# Autodesk Inventor assembly: MR106ZZ1
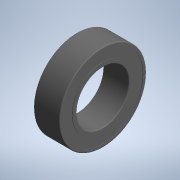
[picture p0: Inventor's stored thumbnail of the model, 180x180]
Saved by Autodesk Inventor 2022 (Build 260153000, 153)
## iProperties
Category: PARTsolutions
Company: NSK_RB
Part Number: MR106ZZ1
Catalog Web Link: www.cadenas.de
Description: Shielded Type ZZ-ZZS-
Vendor: NSK_RB
Document SubType Name: Assembly
Designer: partserver
Manufacturer: NSK_RB
Mass: 0.68 g
Surface Area: 5.5525 cm^2
Volume: 0.0980642 cm^3
Density: 6.93423 g/cm^3
PSOL_IDENT_0: {$CADENAS_DATA\23d-libs\nsk_rb\roller_bearings\deep_groove_bb\exstra_small_miniatur_bb\metric_design
PSOL_IDENT_1: \shielded_type_zz_zzs_asmtab.prj},176 {VTYP=3D},{STYP=ASSTAB},{NB=MR106ZZ1},{LINA=MR106ZZ1},{NN=Shie
PSOL_IDENT_2: lded Type ZZ-ZZS},{DATE=25.05.2021 06:41:25},{GEOMDATE=14.01.2008},{VERSION=},{LINEID=600},{WBVAR=},
PSOL_IDENT_3: {WBNUMERIC=}  {NB=MR106ZZ1},{LINA=MR106ZZ1},{KT=DUMMY},{IDNR=},{STAN=Standard},{ORDER=MR106ZZ1},{SD=
PSOL_IDENT_4: 6.0},{X=6.0},{DI1=7.04},{DI2=7.04},{SDE1=8.90},{SDE2=9.25},{D=10},{DD=10},{B=0.0},{B1=3.0},{R=0.00},
PSOL_IDENT_5: {R1=0.10},{CR1=495},{COR1=218},{CR2=51},{COR2=22.0},{LG=45000},{LO=53000},{DA=0.0},{DB=7.0},{DA1=0.0
PSOL_IDENT_6: },{DB1=9.3},{RA=0.00},{RB=0.10},{MASS=0.68},{SC=1},{PPATH=shielded_type_zz_zzs_asmtpl.prj}
NB: MR106ZZ1
NN: Shielded Type ZZ-ZZS
NBSYN: $ORDER.
LINA: MR106ZZ1
CATALOG: NSK Rolling Bearing
STAN: Standard
ORDER: MR106ZZ1
SD: 6
D: 10
B1: 3
R1: 0.1
CR1: 495
COR1: 218
CR2: 51
COR2: 22
LG: 45000
DB: 7
DB1: 9.3
RB: 0.1
MASS: 0.68
SUPPLIER: NSK_RB
ARTICLENO: MR106ZZ1
BOMINFO: MR106ZZ1
CREATOR: CADENAS GmbH
Title: MR106ZZ1
Author: Cadenas PARTsolutions
## Documents named in this file (6)
- C:\Users\rkawaba1\Documents\GrabCAD\NHK2022\BasicParts\Bearing\MR106ZZ1\MR106ZZ1.iam
- C:\Users\rkawaba1\Documents\GrabCAD\NHK2022\BasicParts\Bearing\MR106ZZ1\MR106ZZ1 Outer Ring.ipt
- C:\Users\rkawaba1\Documents\GrabCAD\NHK2022\BasicParts\Bearing\MR106ZZ1\MR106ZZ1 Inner Ring.ipt
- C:\Users\rkawaba1\Documents\GrabCAD\NHK2022\BasicParts\Bearing\MR106ZZ1\MR106ZZ1 Shield1.ipt
- C:\Users\rkawaba1\Documents\GrabCAD\NHK2022\BasicParts\Bearing\MR106ZZ1\MR106ZZ1 Ball.ipt
- C:\Users\rkawaba1\Documents\GrabCAD\NHK2022\BasicParts\Bearing\MR106ZZ1\MR106ZZ1 Shield2.ipt
## Components (20 placed, 5 different names)
1. MR106ZZ1 Outer Ring:1 — ip_st_or_1_XY@1 <-> ip_st_ir_1a_XY@2, ip_st_or_1_Z@1 <-> ip_st_ir_1a_Z@2, ip_st_or_1_YZ@1 <-> ip_st_ir_1a_YZ@2, ip_st_or_2_XY@1 <-> ip_st_s2_XY@20, ip_st_or_2_Z@1 <-> ip_st_s2_Z@20, ip_st_or_2_YZ@1 <-> ip_st_s2_YZ@20
2. MR106ZZ1 Inner Ring:1 — ip_st_or_1_XY@1 <-> ip_st_ir_1a_XY@2, ip_st_or_1_Z@1 <-> ip_st_ir_1a_Z@2, ip_st_or_1_YZ@1 <-> ip_st_ir_1a_YZ@2, ip_st_ir_2a_XY@2 <-> ip_st_s1_XY@3, ip_st_ir_2a_Z@2 <-> ip_st_s1_Z@3, ip_st_ir_2a_YZ@2 <-> ip_st_s1_YZ@3, ip_st_ir_1_1_XY@2 <-> ip_st_b_XY@4, ip_st_ir_1_1_Z@2 <-> ip_st_b_Z@4, ip_st_ir_1_1_YZ@2 <-> ip_st_b_YZ@4, ip_st_ir_1_2_XY@2 <-> ip_st_b_XY@5, ip_st_ir_1_2_Z@2 <-> ip_st_b_Z@5, ip_st_ir_1_2_YZ@2 <-> ip_st_b_YZ@5, ip_st_ir_1_3_XY@2 <-> ip_st_b_XY@6, ip_st_ir_1_3_Z@2 <-> ip_st_b_Z@6, ip_st_ir_1_3_YZ@2 <-> ip_st_b_YZ@6, ip_st_ir_1_4_XY@2 <-> ip_st_b_XY@7, ip_st_ir_1_4_Z@2 <-> ip_st_b_Z@7, ip_st_ir_1_4_YZ@2 <-> ip_st_b_YZ@7, ip_st_ir_1_5_XY@2 <-> ip_st_b_XY@8, ip_st_ir_1_5_Z@2 <-> ip_st_b_Z@8, ip_st_ir_1_5_YZ@2 <-> ip_st_b_YZ@8, ip_st_ir_1_6_XY@2 <-> ip_st_b_XY@9, ip_st_ir_1_6_Z@2 <-> ip_st_b_Z@9, ip_st_ir_1_6_YZ@2 <-> ip_st_b_YZ@9, ip_st_ir_1_7_XY@2 <-> ip_st_b_XY@10, ip_st_ir_1_7_Z@2 <-> ip_st_b_Z@10, ip_st_ir_1_7_YZ@2 <-> ip_st_b_YZ@10, ip_st_ir_1_8_XY@2 <-> ip_st_b_XY@11, ip_st_ir_1_8_Z@2 <-> ip_st_b_Z@11, ip_st_ir_1_8_YZ@2 <-> ip_st_b_YZ@11, ip_st_ir_1_9_XY@2 <-> ip_st_b_XY@12, ip_st_ir_1_9_Z@2 <-> ip_st_b_Z@12, ip_st_ir_1_9_YZ@2 <-> ip_st_b_YZ@12, ip_st_ir_1_10_XY@2 <-> ip_st_b_XY@13, ip_st_ir_1_10_Z@2 <-> ip_st_b_Z@13, ip_st_ir_1_10_YZ@2 <-> ip_st_b_YZ@13, ip_st_ir_1_11_XY@2 <-> ip_st_b_XY@14, ip_st_ir_1_11_Z@2 <-> ip_st_b_Z@14, ip_st_ir_1_11_YZ@2 <-> ip_st_b_YZ@14, ip_st_ir_1_12_XY@2 <-> ip_st_b_XY@15, ip_st_ir_1_12_Z@2 <-> ip_st_b_Z@15, ip_st_ir_1_12_YZ@2 <-> ip_st_b_YZ@15, ip_st_ir_1_13_XY@2 <-> ip_st_b_XY@16, ip_st_ir_1_13_Z@2 <-> ip_st_b_Z@16, ip_st_ir_1_13_YZ@2 <-> ip_st_b_YZ@16, ip_st_ir_1_14_XY@2 <-> ip_st_b_XY@17, ip_st_ir_1_14_Z@2 <-> ip_st_b_Z@17, ip_st_ir_1_14_YZ@2 <-> ip_st_b_YZ@17, ip_st_ir_1_15_XY@2 <-> ip_st_b_XY@18, ip_st_ir_1_15_Z@2 <-> ip_st_b_Z@18, ip_st_ir_1_15_YZ@2 <-> ip_st_b_YZ@18, ip_st_ir_1_16_XY@2 <-> ip_st_b_XY@19, ip_st_ir_1_16_Z@2 <-> ip_st_b_Z@19, ip_st_ir_1_16_YZ@2 <-> ip_st_b_YZ@19
3. MR106ZZ1 Shield1:1 — ip_st_ir_2a_XY@2 <-> ip_st_s1_XY@3, ip_st_ir_2a_Z@2 <-> ip_st_s1_Z@3, ip_st_ir_2a_YZ@2 <-> ip_st_s1_YZ@3
4. MR106ZZ1 Ball:1 — ip_st_ir_1_1_XY@2 <-> ip_st_b_XY@4, ip_st_ir_1_1_Z@2 <-> ip_st_b_Z@4, ip_st_ir_1_1_YZ@2 <-> ip_st_b_YZ@4
5. MR106ZZ1 Ball:2 — ip_st_ir_1_2_XY@2 <-> ip_st_b_XY@5, ip_st_ir_1_2_Z@2 <-> ip_st_b_Z@5, ip_st_ir_1_2_YZ@2 <-> ip_st_b_YZ@5
6. MR106ZZ1 Ball:3 — ip_st_ir_1_3_XY@2 <-> ip_st_b_XY@6, ip_st_ir_1_3_Z@2 <-> ip_st_b_Z@6, ip_st_ir_1_3_YZ@2 <-> ip_st_b_YZ@6
7. MR106ZZ1 Ball:4 — ip_st_ir_1_4_XY@2 <-> ip_st_b_XY@7, ip_st_ir_1_4_Z@2 <-> ip_st_b_Z@7, ip_st_ir_1_4_YZ@2 <-> ip_st_b_YZ@7
8. MR106ZZ1 Ball:5 — ip_st_ir_1_5_XY@2 <-> ip_st_b_XY@8, ip_st_ir_1_5_Z@2 <-> ip_st_b_Z@8, ip_st_ir_1_5_YZ@2 <-> ip_st_b_YZ@8
9. MR106ZZ1 Ball:6 — ip_st_ir_1_6_XY@2 <-> ip_st_b_XY@9, ip_st_ir_1_6_Z@2 <-> ip_st_b_Z@9, ip_st_ir_1_6_YZ@2 <-> ip_st_b_YZ@9
10. MR106ZZ1 Ball:7 — ip_st_ir_1_7_XY@2 <-> ip_st_b_XY@10, ip_st_ir_1_7_Z@2 <-> ip_st_b_Z@10, ip_st_ir_1_7_YZ@2 <-> ip_st_b_YZ@10
11. MR106ZZ1 Ball:8 — ip_st_ir_1_8_XY@2 <-> ip_st_b_XY@11, ip_st_ir_1_8_Z@2 <-> ip_st_b_Z@11, ip_st_ir_1_8_YZ@2 <-> ip_st_b_YZ@11
12. MR106ZZ1 Ball:9 — ip_st_ir_1_9_XY@2 <-> ip_st_b_XY@12, ip_st_ir_1_9_Z@2 <-> ip_st_b_Z@12, ip_st_ir_1_9_YZ@2 <-> ip_st_b_YZ@12
13. MR106ZZ1 Ball:10 — ip_st_ir_1_10_XY@2 <-> ip_st_b_XY@13, ip_st_ir_1_10_Z@2 <-> ip_st_b_Z@13, ip_st_ir_1_10_YZ@2 <-> ip_st_b_YZ@13
14. MR106ZZ1 Ball:11 — ip_st_ir_1_11_XY@2 <-> ip_st_b_XY@14, ip_st_ir_1_11_Z@2 <-> ip_st_b_Z@14, ip_st_ir_1_11_YZ@2 <-> ip_st_b_YZ@14
15. MR106ZZ1 Ball:12 — ip_st_ir_1_12_XY@2 <-> ip_st_b_XY@15, ip_st_ir_1_12_Z@2 <-> ip_st_b_Z@15, ip_st_ir_1_12_YZ@2 <-> ip_st_b_YZ@15
16. MR106ZZ1 Ball:13 — ip_st_ir_1_13_XY@2 <-> ip_st_b_XY@16, ip_st_ir_1_13_Z@2 <-> ip_st_b_Z@16, ip_st_ir_1_13_YZ@2 <-> ip_st_b_YZ@16
17. MR106ZZ1 Ball:14 — ip_st_ir_1_14_XY@2 <-> ip_st_b_XY@17, ip_st_ir_1_14_Z@2 <-> ip_st_b_Z@17, ip_st_ir_1_14_YZ@2 <-> ip_st_b_YZ@17
18. MR106ZZ1 Ball:15 — ip_st_ir_1_15_XY@2 <-> ip_st_b_XY@18, ip_st_ir_1_15_Z@2 <-> ip_st_b_Z@18, ip_st_ir_1_15_YZ@2 <-> ip_st_b_YZ@18
19. MR106ZZ1 Ball:16 — ip_st_ir_1_16_XY@2 <-> ip_st_b_XY@19, ip_st_ir_1_16_Z@2 <-> ip_st_b_Z@19, ip_st_ir_1_16_YZ@2 <-> ip_st_b_YZ@19
20. MR106ZZ1 Shield2:1 — ip_st_or_2_XY@1 <-> ip_st_s2_XY@20, ip_st_or_2_Z@1 <-> ip_st_s2_Z@20, ip_st_or_2_YZ@1 <-> ip_st_s2_YZ@20
## Relationships (57: Mate 37, Angle 19, Flush 1)
- ip_st_or_1_XY@1 <-> ip_st_ir_1a_XY@2 [Flush]: MR106ZZ1 Outer Ring:1 ↔ MR106ZZ1 Inner Ring:1
- ip_st_or_1_Z@1 <-> ip_st_ir_1a_Z@2 [Mate]: MR106ZZ1 Outer Ring:1 ↔ MR106ZZ1 Inner Ring:1
- ip_st_or_1_YZ@1 <-> ip_st_ir_1a_YZ@2 [Angle] (90 deg): MR106ZZ1 Outer Ring:1 ↔ MR106ZZ1 Inner Ring:1
- ip_st_ir_2a_XY@2 <-> ip_st_s1_XY@3 [Mate]: MR106ZZ1 Inner Ring:1 ↔ MR106ZZ1 Shield1:1
- ip_st_ir_2a_Z@2 <-> ip_st_s1_Z@3 [Mate]: MR106ZZ1 Inner Ring:1 ↔ MR106ZZ1 Shield1:1
- ip_st_ir_2a_YZ@2 <-> ip_st_s1_YZ@3 [Angle] (0 deg): MR106ZZ1 Inner Ring:1 ↔ MR106ZZ1 Shield1:1
- ip_st_ir_1_1_XY@2 <-> ip_st_b_XY@4 [Mate]: MR106ZZ1 Inner Ring:1 ↔ MR106ZZ1 Ball:1
- ip_st_ir_1_1_Z@2 <-> ip_st_b_Z@4 [Mate]: MR106ZZ1 Inner Ring:1 ↔ MR106ZZ1 Ball:1
- ip_st_ir_1_1_YZ@2 <-> ip_st_b_YZ@4 [Angle] (0 deg): MR106ZZ1 Inner Ring:1 ↔ MR106ZZ1 Ball:1
- ip_st_ir_1_2_XY@2 <-> ip_st_b_XY@5 [Mate]: MR106ZZ1 Inner Ring:1 ↔ MR106ZZ1 Ball:2
- ip_st_ir_1_2_Z@2 <-> ip_st_b_Z@5 [Mate]: MR106ZZ1 Inner Ring:1 ↔ MR106ZZ1 Ball:2
- ip_st_ir_1_2_YZ@2 <-> ip_st_b_YZ@5 [Angle] (0 deg): MR106ZZ1 Inner Ring:1 ↔ MR106ZZ1 Ball:2
- ip_st_ir_1_3_XY@2 <-> ip_st_b_XY@6 [Mate]: MR106ZZ1 Inner Ring:1 ↔ MR106ZZ1 Ball:3
- ip_st_ir_1_3_Z@2 <-> ip_st_b_Z@6 [Mate]: MR106ZZ1 Inner Ring:1 ↔ MR106ZZ1 Ball:3
- ip_st_ir_1_3_YZ@2 <-> ip_st_b_YZ@6 [Angle] (0 deg): MR106ZZ1 Inner Ring:1 ↔ MR106ZZ1 Ball:3
- ip_st_ir_1_4_XY@2 <-> ip_st_b_XY@7 [Mate]: MR106ZZ1 Inner Ring:1 ↔ MR106ZZ1 Ball:4
- ip_st_ir_1_4_Z@2 <-> ip_st_b_Z@7 [Mate]: MR106ZZ1 Inner Ring:1 ↔ MR106ZZ1 Ball:4
- ip_st_ir_1_4_YZ@2 <-> ip_st_b_YZ@7 [Angle] (0 deg): MR106ZZ1 Inner Ring:1 ↔ MR106ZZ1 Ball:4
- ip_st_ir_1_5_XY@2 <-> ip_st_b_XY@8 [Mate]: MR106ZZ1 Inner Ring:1 ↔ MR106ZZ1 Ball:5
- ip_st_ir_1_5_Z@2 <-> ip_st_b_Z@8 [Mate]: MR106ZZ1 Inner Ring:1 ↔ MR106ZZ1 Ball:5
- ip_st_ir_1_5_YZ@2 <-> ip_st_b_YZ@8 [Angle] (0 deg): MR106ZZ1 Inner Ring:1 ↔ MR106ZZ1 Ball:5
- ip_st_ir_1_6_XY@2 <-> ip_st_b_XY@9 [Mate]: MR106ZZ1 Inner Ring:1 ↔ MR106ZZ1 Ball:6
- ip_st_ir_1_6_Z@2 <-> ip_st_b_Z@9 [Mate]: MR106ZZ1 Inner Ring:1 ↔ MR106ZZ1 Ball:6
- ip_st_ir_1_6_YZ@2 <-> ip_st_b_YZ@9 [Angle] (0 deg): MR106ZZ1 Inner Ring:1 ↔ MR106ZZ1 Ball:6
- ip_st_ir_1_7_XY@2 <-> ip_st_b_XY@10 [Mate]: MR106ZZ1 Inner Ring:1 ↔ MR106ZZ1 Ball:7
- ip_st_ir_1_7_Z@2 <-> ip_st_b_Z@10 [Mate]: MR106ZZ1 Inner Ring:1 ↔ MR106ZZ1 Ball:7
- ip_st_ir_1_7_YZ@2 <-> ip_st_b_YZ@10 [Angle] (0 deg): MR106ZZ1 Inner Ring:1 ↔ MR106ZZ1 Ball:7
- ip_st_ir_1_8_XY@2 <-> ip_st_b_XY@11 [Mate]: MR106ZZ1 Inner Ring:1 ↔ MR106ZZ1 Ball:8
- ip_st_ir_1_8_Z@2 <-> ip_st_b_Z@11 [Mate]: MR106ZZ1 Inner Ring:1 ↔ MR106ZZ1 Ball:8
- ip_st_ir_1_8_YZ@2 <-> ip_st_b_YZ@11 [Angle] (0 deg): MR106ZZ1 Inner Ring:1 ↔ MR106ZZ1 Ball:8
- ip_st_ir_1_9_XY@2 <-> ip_st_b_XY@12 [Mate]: MR106ZZ1 Inner Ring:1 ↔ MR106ZZ1 Ball:9
- ip_st_ir_1_9_Z@2 <-> ip_st_b_Z@12 [Mate]: MR106ZZ1 Inner Ring:1 ↔ MR106ZZ1 Ball:9
- ip_st_ir_1_9_YZ@2 <-> ip_st_b_YZ@12 [Angle] (0 deg): MR106ZZ1 Inner Ring:1 ↔ MR106ZZ1 Ball:9
- ip_st_ir_1_10_XY@2 <-> ip_st_b_XY@13 [Mate]: MR106ZZ1 Inner Ring:1 ↔ MR106ZZ1 Ball:10
- ip_st_ir_1_10_Z@2 <-> ip_st_b_Z@13 [Mate]: MR106ZZ1 Inner Ring:1 ↔ MR106ZZ1 Ball:10
- ip_st_ir_1_10_YZ@2 <-> ip_st_b_YZ@13 [Angle] (0 deg): MR106ZZ1 Inner Ring:1 ↔ MR106ZZ1 Ball:10
- ip_st_ir_1_11_XY@2 <-> ip_st_b_XY@14 [Mate]: MR106ZZ1 Inner Ring:1 ↔ MR106ZZ1 Ball:11
- ip_st_ir_1_11_Z@2 <-> ip_st_b_Z@14 [Mate]: MR106ZZ1 Inner Ring:1 ↔ MR106ZZ1 Ball:11
- ip_st_ir_1_11_YZ@2 <-> ip_st_b_YZ@14 [Angle] (0 deg): MR106ZZ1 Inner Ring:1 ↔ MR106ZZ1 Ball:11
- ip_st_ir_1_12_XY@2 <-> ip_st_b_XY@15 [Mate]: MR106ZZ1 Inner Ring:1 ↔ MR106ZZ1 Ball:12
- ip_st_ir_1_12_Z@2 <-> ip_st_b_Z@15 [Mate]: MR106ZZ1 Inner Ring:1 ↔ MR106ZZ1 Ball:12
- ip_st_ir_1_12_YZ@2 <-> ip_st_b_YZ@15 [Angle] (0 deg): MR106ZZ1 Inner Ring:1 ↔ MR106ZZ1 Ball:12
- ip_st_ir_1_13_XY@2 <-> ip_st_b_XY@16 [Mate]: MR106ZZ1 Inner Ring:1 ↔ MR106ZZ1 Ball:13
- ip_st_ir_1_13_Z@2 <-> ip_st_b_Z@16 [Mate]: MR106ZZ1 Inner Ring:1 ↔ MR106ZZ1 Ball:13
- ip_st_ir_1_13_YZ@2 <-> ip_st_b_YZ@16 [Angle] (0 deg): MR106ZZ1 Inner Ring:1 ↔ MR106ZZ1 Ball:13
- ip_st_ir_1_14_XY@2 <-> ip_st_b_XY@17 [Mate]: MR106ZZ1 Inner Ring:1 ↔ MR106ZZ1 Ball:14
- ip_st_ir_1_14_Z@2 <-> ip_st_b_Z@17 [Mate]: MR106ZZ1 Inner Ring:1 ↔ MR106ZZ1 Ball:14
- ip_st_ir_1_14_YZ@2 <-> ip_st_b_YZ@17 [Angle] (0 deg): MR106ZZ1 Inner Ring:1 ↔ MR106ZZ1 Ball:14
- ip_st_ir_1_15_XY@2 <-> ip_st_b_XY@18 [Mate]: MR106ZZ1 Inner Ring:1 ↔ MR106ZZ1 Ball:15
- ip_st_ir_1_15_Z@2 <-> ip_st_b_Z@18 [Mate]: MR106ZZ1 Inner Ring:1 ↔ MR106ZZ1 Ball:15
- ip_st_ir_1_15_YZ@2 <-> ip_st_b_YZ@18 [Angle] (0 deg): MR106ZZ1 Inner Ring:1 ↔ MR106ZZ1 Ball:15
- ip_st_ir_1_16_XY@2 <-> ip_st_b_XY@19 [Mate]: MR106ZZ1 Inner Ring:1 ↔ MR106ZZ1 Ball:16
- ip_st_ir_1_16_Z@2 <-> ip_st_b_Z@19 [Mate]: MR106ZZ1 Inner Ring:1 ↔ MR106ZZ1 Ball:16
- ip_st_ir_1_16_YZ@2 <-> ip_st_b_YZ@19 [Angle] (0 deg): MR106ZZ1 Inner Ring:1 ↔ MR106ZZ1 Ball:16
- ip_st_or_2_XY@1 <-> ip_st_s2_XY@20 [Mate]: MR106ZZ1 Outer Ring:1 ↔ MR106ZZ1 Shield2:1
- ip_st_or_2_Z@1 <-> ip_st_s2_Z@20 [Mate]: MR106ZZ1 Outer Ring:1 ↔ MR106ZZ1 Shield2:1
- ip_st_or_2_YZ@1 <-> ip_st_s2_YZ@20 [Angle] (0 deg): MR106ZZ1 Outer Ring:1 ↔ MR106ZZ1 Shield2:1
